# Autodesk Inventor assembly: Subensamble_Base cortadora_MIR
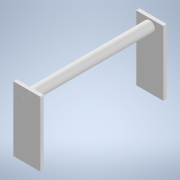
[picture p0: Inventor's stored thumbnail of the model, 180x180]
Saved by Autodesk Inventor 2021 (Build 250183000, 183)
## iProperties
Created: 2021-04-30
Part Number: Subensamble_Base cortadora_MIR
Document SubType Name: Assembly
Designer: maaro
Author: Admin
## Documents named in this file (3)
- C:\Users\Nelson\Github\Proyecto_APM\Inventor_Corte\Subensamble_Base cortadora_MIR.iam
- C:\Users\Nelson\Github\Proyecto_APM\Inventor_Corte\Base_cortadora_MIR.ipt
- C:\Users\Nelson\Github\Proyecto_APM\Inventor_Corte\Barra base cotadora_MIR.ipt
## Components (3 placed, 2 different names)
1. Base_cortadora_MIR:1 — Flush:2, Mate:2
2. Base_cortadora_MIR:2 — Flush:2, Mate:1
3. Barra base cotadora_MIR:1 — Flush:2, Mate:1, Flush:2, Mate:2
## Relationships (4: Flush 2, Mate 2)
- Flush:2: Base_cortadora_MIR:2 ↔ Barra base cotadora_MIR:1
- Mate:1: Base_cortadora_MIR:2 ↔ Barra base cotadora_MIR:1
- Flush:2: Base_cortadora_MIR:1 ↔ Barra base cotadora_MIR:1
- Mate:2: Base_cortadora_MIR:1 ↔ Barra base cotadora_MIR:1
